# Autodesk Inventor assembly: 04-RecombinationToDetector
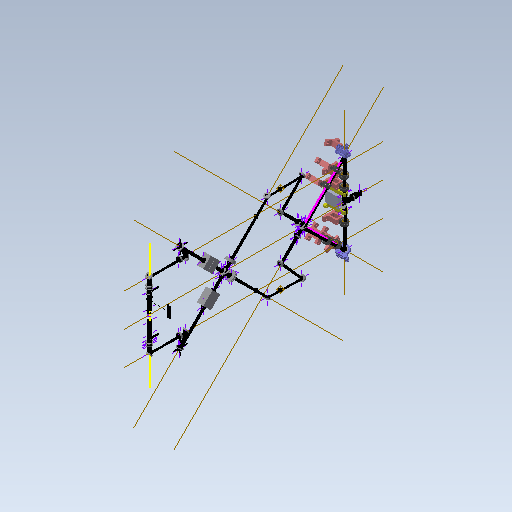
[picture p0: Inventor's stored thumbnail of the model, 512x512]
Saved by Autodesk Inventor 2020 (Build 240168000, 168)
## iProperties
Created: 2016-12-02
Part Number: 04-RecombinationToDetector
Document SubType Name: Assembly
Designer: map
Author: map
## Documents named in this file (7)
- C:\Users\whgu0532\Documents\4Pi\4Pi-Oxford\04-RecombinationToDetector.iam
- C:\Users\whgu0532\Documents\4Pi\4Pi-Oxford\SS100-F3H.ipt
- C:\Users\whgu0532\Documents\4Pi\4Pi-Oxford\FAB-P0019 - Mirror Mount, SS100.ipt
- C:\Users\whgu0532\Documents\4Pi\4Pi-Oxford\__CAVITY_AND_IMAGING_OPTICS__.iam
- C:\Users\whgu0532\Documents\4Pi\4Pi-Oxford\FAB-P0039 - Combining Mirror Mt.ipt
- C:\Users\whgu0532\Documents\4Pi\4Pi-Oxford\Alignment Assembly after Cavity.iam
- C:\Users\whgu0532\Documents\4Pi\4Pi-Oxford\FAB-OX0015-LensMount-15mm-epoxied.ipt
## Components (15 placed, 12 different names)
1. __CAVITY_AND_IMAGING_OPTICS__:1 [sub-assembly] — Angle:1, Angle:2, Mate:7, Mate:8, Mate:9, Mate:10, Tangent:2, Mate:11, Mate:12, Mate:16, Mate:17, Mate:18, Mate:19, Mate:20, Mate:21, Mate:22, Mate:23, Mate:24, Angle:8, Angle:9, Tangent:3, Mate:26, Tangent:4, Mate:27, Tangent:5
2. SS100-F3H:1 — Mate:1, Mate:8, Mate:27, Tangent:5
3. FAB-P0019 - Mirror Mount, SS100:1 — Mate:1, Angle:1, Flush:1
4. SS100-F3H:3 — Mate:4, Mate:7, Mate:26, Tangent:4
5. FAB-P0019 - Mirror Mount, SS100:2 — Mate:4, Angle:2, Flush:1, Angle:3, Flush:2, Flush:3, Flush:4, Flush:5, Flush:6, Flush:7, Flush:8, Flush:9, Flush:11, Flush:12
6. FAB-P0039 - Combining Mirror Mt:1 — Mate:9, Mate:10, Flush:2, Angle:10, Angle:12, Angle:14
7. FAB-OX0015-LensMount-15mm-epoxied:1 — Flush:3, Mate:12, Tangent:3
8. FAB-OX0015-LensMount-15mm-epoxied:2 — Flush:4, Tangent:2, Mate:11
9. Alignment Assembly after Cavity:UpperTransmitted1 [sub-assembly] — Flush:5, Mate:19, Angle:7, Angle:8, Symmetry:1, Angle:15
10. Alignment Assembly after Cavity:UpperReflected1 [sub-assembly] — Flush:6, Mate:20, Angle:7, Symmetry:2, Angle:15
11. Alignment Assembly after Cavity:UpperTransmitted2 [sub-assembly] — Flush:12, Mate:22, Angle:6, Angle:9, Angle:13
12. Alignment Assembly after Cavity:UpperReflected2 [sub-assembly] — Flush:11, Mate:21, Angle:6, Angle:13, Angle:14
13. Alignment Assembly after Cavity:LowerTransmitted1 [sub-assembly] — Flush:8, Mate:18, Angle:4, Symmetry:2, Angle:11
14. Alignment Assembly after Cavity:LowerReflected1 [sub-assembly] — Flush:7, Mate:17, Angle:4, Symmetry:1, Angle:11
15. Alignment Assembly after Cavity:LowerTransmitted2 [sub-assembly] — Flush:9, Mate:16, Mate:25, Angle:10, Angle:12
## Relationships (55: Mate 24, Angle 14, Flush 11, Tangent 4, Symmetry 2)
- Mate:1: SS100-F3H:1 ↔ FAB-P0019 - Mirror Mount, SS100:1
- [Mate]: SS100-F3H:1 ↔ FAB-P0019 - Mirror Mount, SS100:1
- [Mate]: SS100-F3H:1 ↔ FAB-P0019 - Mirror Mount, SS100:1
- Mate:4: SS100-F3H:3 ↔ FAB-P0019 - Mirror Mount, SS100:2
- [Mate]: SS100-F3H:3 ↔ FAB-P0019 - Mirror Mount, SS100:2
- [Mate]: SS100-F3H:3 ↔ FAB-P0019 - Mirror Mount, SS100:2
- Angle:1 (0 deg): __CAVITY_AND_IMAGING_OPTICS__:1 ↔ FAB-P0019 - Mirror Mount, SS100:1
- Angle:2 (0 deg): __CAVITY_AND_IMAGING_OPTICS__:1 ↔ FAB-P0019 - Mirror Mount, SS100:2
- Flush:1: FAB-P0019 - Mirror Mount, SS100:1 ↔ FAB-P0019 - Mirror Mount, SS100:2
- Mate:7: __CAVITY_AND_IMAGING_OPTICS__:1 ↔ SS100-F3H:3
- Mate:8: __CAVITY_AND_IMAGING_OPTICS__:1 ↔ SS100-F3H:1
- Angle:3 (180 deg): FAB-P0019 - Mirror Mount, SS100:2
- Mate:9: __CAVITY_AND_IMAGING_OPTICS__:1 ↔ FAB-P0039 - Combining Mirror Mt:1
- Mate:10: __CAVITY_AND_IMAGING_OPTICS__:1 ↔ FAB-P0039 - Combining Mirror Mt:1
- Flush:2: FAB-P0019 - Mirror Mount, SS100:2 ↔ FAB-P0039 - Combining Mirror Mt:1
- Flush:3: FAB-P0019 - Mirror Mount, SS100:2 ↔ FAB-OX0015-LensMount-15mm-epoxied:1
- Flush:4: FAB-P0019 - Mirror Mount, SS100:2 ↔ FAB-OX0015-LensMount-15mm-epoxied:2
- Tangent:2 (-0.375 mm): __CAVITY_AND_IMAGING_OPTICS__:1 ↔ FAB-OX0015-LensMount-15mm-epoxied:2
- Mate:11: __CAVITY_AND_IMAGING_OPTICS__:1 ↔ FAB-OX0015-LensMount-15mm-epoxied:2
- Mate:12: __CAVITY_AND_IMAGING_OPTICS__:1 ↔ FAB-OX0015-LensMount-15mm-epoxied:1
- Flush:5: FAB-P0019 - Mirror Mount, SS100:2 ↔ Alignment Assembly after Cavity:UpperTransmitted1
- Flush:6: FAB-P0019 - Mirror Mount, SS100:2 ↔ Alignment Assembly after Cavity:UpperReflected1
- Flush:7: FAB-P0019 - Mirror Mount, SS100:2 ↔ Alignment Assembly after Cavity:LowerReflected1
- Flush:8: FAB-P0019 - Mirror Mount, SS100:2 ↔ Alignment Assembly after Cavity:LowerTransmitted1
- Flush:9: FAB-P0019 - Mirror Mount, SS100:2 ↔ Alignment Assembly after Cavity:LowerTransmitted2
- Flush:11: FAB-P0019 - Mirror Mount, SS100:2 ↔ Alignment Assembly after Cavity:UpperReflected2
- Flush:12: FAB-P0019 - Mirror Mount, SS100:2 ↔ Alignment Assembly after Cavity:UpperTransmitted2
- Mate:16: __CAVITY_AND_IMAGING_OPTICS__:1 ↔ Alignment Assembly after Cavity:LowerTransmitted2
- Mate:17: __CAVITY_AND_IMAGING_OPTICS__:1 ↔ Alignment Assembly after Cavity:LowerReflected1
- Mate:18: __CAVITY_AND_IMAGING_OPTICS__:1 ↔ Alignment Assembly after Cavity:LowerTransmitted1
- Mate:19: __CAVITY_AND_IMAGING_OPTICS__:1 ↔ Alignment Assembly after Cavity:UpperTransmitted1
- Mate:20: __CAVITY_AND_IMAGING_OPTICS__:1 ↔ Alignment Assembly after Cavity:UpperReflected1
- Mate:21: __CAVITY_AND_IMAGING_OPTICS__:1 ↔ Alignment Assembly after Cavity:UpperReflected2
- Mate:22: __CAVITY_AND_IMAGING_OPTICS__:1 ↔ Alignment Assembly after Cavity:UpperTransmitted2
- Angle:4 (0 deg): Alignment Assembly after Cavity:LowerTransmitted1 ↔ Alignment Assembly after Cavity:LowerReflected1
- Angle:6 (0 deg): Alignment Assembly after Cavity:UpperTransmitted2 ↔ Alignment Assembly after Cavity:UpperReflected2
- Angle:7 (0 deg): Alignment Assembly after Cavity:UpperTransmitted1 ↔ Alignment Assembly after Cavity:UpperReflected1
- Mate:23: __CAVITY_AND_IMAGING_OPTICS__:1
- Mate:24: __CAVITY_AND_IMAGING_OPTICS__:1
- Mate:25: Alignment Assembly after Cavity:LowerTransmitted2
- Angle:8 (0 deg): __CAVITY_AND_IMAGING_OPTICS__:1 ↔ Alignment Assembly after Cavity:UpperTransmitted1
- Angle:9 (0 deg): __CAVITY_AND_IMAGING_OPTICS__:1 ↔ Alignment Assembly after Cavity:UpperTransmitted2
- Angle:10 (180 deg): FAB-P0039 - Combining Mirror Mt:1 ↔ Alignment Assembly after Cavity:LowerTransmitted2
- Symmetry:1: Alignment Assembly after Cavity:UpperTransmitted1 ↔ Alignment Assembly after Cavity:LowerReflected1
- Symmetry:2: Alignment Assembly after Cavity:UpperReflected1 ↔ Alignment Assembly after Cavity:LowerTransmitted1
- Tangent:3 (-0.375 mm): __CAVITY_AND_IMAGING_OPTICS__:1 ↔ FAB-OX0015-LensMount-15mm-epoxied:1
- Angle:11 (0 deg): Alignment Assembly after Cavity:LowerTransmitted1 ↔ Alignment Assembly after Cavity:LowerReflected1
- Angle:12 (0 deg): FAB-P0039 - Combining Mirror Mt:1 ↔ Alignment Assembly after Cavity:LowerTransmitted2
- Angle:13 (0 deg): Alignment Assembly after Cavity:UpperTransmitted2 ↔ Alignment Assembly after Cavity:UpperReflected2
- Angle:14 (0 deg): FAB-P0039 - Combining Mirror Mt:1 ↔ Alignment Assembly after Cavity:UpperReflected2
- Angle:15 (0 deg): Alignment Assembly after Cavity:UpperTransmitted1 ↔ Alignment Assembly after Cavity:UpperReflected1
- Mate:26: __CAVITY_AND_IMAGING_OPTICS__:1 ↔ SS100-F3H:3
- Tangent:4: __CAVITY_AND_IMAGING_OPTICS__:1 ↔ SS100-F3H:3
- Mate:27: __CAVITY_AND_IMAGING_OPTICS__:1 ↔ SS100-F3H:1
- Tangent:5: __CAVITY_AND_IMAGING_OPTICS__:1 ↔ SS100-F3H:1
## Named parameters: d15_d10 = 0.2 mm, d16_d11 = 0 mm, d17_d12 = 0 mm, d18_d13 = 0 mm, d19_d9 = 0 mm, d40_d38 = 0 mm, d41_d39 = 0 mm, d42_d29_d10 = 0.2 mm, d43_d30_d11 = 0 mm, d44_d31_d12 = 0 mm, d45_d32_d13 = 0 mm, d46_d33_d9 = 0 mm
